# Autodesk Inventor assembly: Assembly1
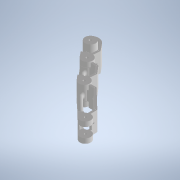
[picture p0: Inventor's stored thumbnail of the model, 180x180]
Saved by Autodesk Inventor 2021 (Build 250183000, 183)
## iProperties
Created: 2022-09-07
Part Number: Assembly1
Document SubType Name: Assembly
Designer: ereg140
Author: ereg140
## Documents named in this file (4)
- \\files.auckland.ac.nz\myhome\Documents\GitHub\hand\PRINTS\Finger3\Assembly1.iam
- \\files.auckland.ac.nz\myhome\Documents\GitHub\hand\Phalalnge3_28mm.ipt
- \\files.auckland.ac.nz\myhome\Documents\GitHub\hand\Phalalnge3_20mm.ipt
- \\files.auckland.ac.nz\myhome\Documents\GitHub\hand\Phalalnge3_42mm.ipt
## Components (3 placed, 3 different names)
1. Phalalnge3_20mm:1 — Rotational:2
2. Phalalnge3_28mm:1 — Rotational:1, Rotational:2
3. Phalalnge3_42mm:1 — Rotational:1
## Relationships (2: RevoluteJoint 2)
- Rotational:1 [RevoluteJoint]: Phalalnge3_28mm:1 ↔ Phalalnge3_42mm:1
- Rotational:2 [RevoluteJoint]: Phalalnge3_20mm:1 ↔ Phalalnge3_28mm:1
